# Autodesk Inventor assembly: HUB ASSEMBLY
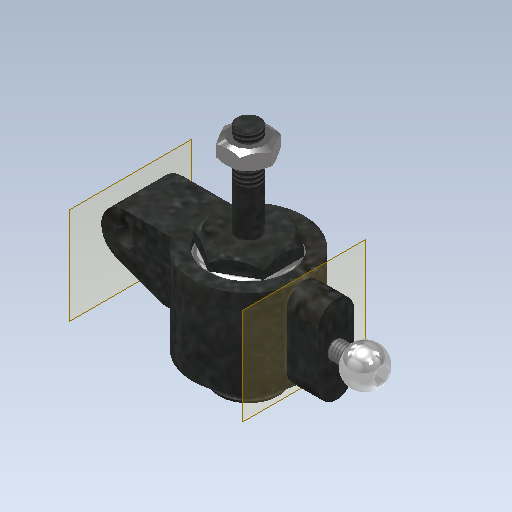
[picture p0: Inventor's stored thumbnail of the model, 512x512]
Saved by Autodesk Inventor 2020 (Build 240168000, 168)
## iProperties
Created: 2015-04-18
Part Number: HUB ASSEMBLY
Document SubType Name: Assembly
Designer: Station9
Author: Station9
## Documents named in this file (6)
- C:\Users\0x6f736f646f\Downloads\rc-car-16.snapshot.3\HUB ASSEMBLY.iam
- C:\Users\0x6f736f646f\Downloads\rc-car-16.snapshot.3\500-126.ipt
- C:\Users\0x6f736f646f\Downloads\rc-car-16.snapshot.3\500-007.ipt
- C:\Users\0x6f736f646f\Downloads\rc-car-16.snapshot.3\500-113.ipt
- C:\Users\0x6f736f646f\Downloads\rc-car-16.snapshot.3\ISO 3245 - 21 D - 10 x 14 x 7(1) I.ipt
- C:\Users\0x6f736f646f\Downloads\rc-car-16.snapshot.3\ISO 4032 - M4ISO.ipt
## Components (5 placed, 5 different names)
1. 500-126:1 — Mate:1, Mate:7, Flush:1, Mate:9
2. 500-007:1 — Mate:1, Mate:4, Mate:6, Mate:8, Mate:9
3. 500-113:1 — Mate:4, Mate:6
4. ISO 3245 (I) 21 D - 10 x 14 x 7:1 — Mate:8
5. ISO 4032 M4:1 — Mate:7, Flush:1
## Relationships (7: Mate 6, Flush 1)
- Mate:1: 500-126:1 ↔ 500-007:1
- Mate:4: 500-007:1 ↔ 500-113:1
- Mate:6 (2.9 mm): 500-007:1 ↔ 500-113:1
- Mate:7: 500-126:1 ↔ ISO 4032 M4:1
- Flush:1 (1.6 mm): 500-126:1 ↔ ISO 4032 M4:1
- Mate:8: 500-007:1 ↔ ISO 3245 (I) 21 D - 10 x 14 x 7:1
- Mate:9: 500-126:1 ↔ 500-007:1
